# Autodesk Inventor assembly: Tête
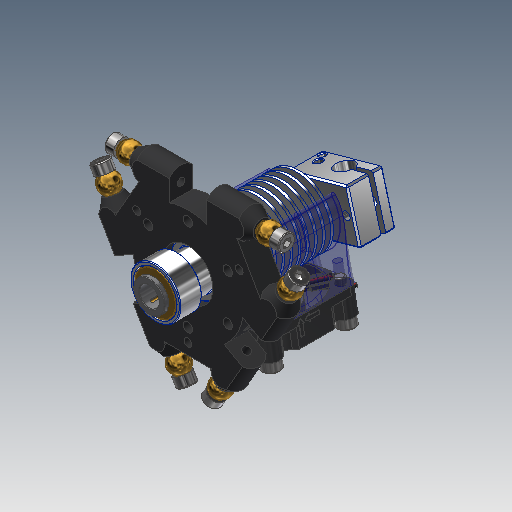
[picture p0: Inventor's stored thumbnail of the model, 512x512]
Saved by Autodesk Inventor 2017 (Build 210142000, 142)
## iProperties
Company: FABLAB Frenchmakers
Part Number: Tête
Material: Générique
Document SubType Name: Assembly
Designer: FABLAB Frenchmakers
Mass: 87.2442 g
Surface Area: 323.979 cm^2
Volume: 30.3794 cm^3
Density: 2.87182 g/cm^3
Project: 1420 Vauban 3D XL
Catalog Web Link: http://frenchmakers.com/
Stock Number: 1420-02-00
## Documents named in this file (8)
- W:\Professionnel\Conception FABLAB\1420-Vauban 3D XL\1420-02 Tete\1420-02-00 Tete.iam
- W:\Professionnel\Conception FABLAB\1420-Vauban 3D XL\1420-02 Tete\1420-02-01 Efflector.ipt
- Support_buse.ipt
- W:\Professionnel\Conception FABLAB\1420-Vauban 3D XL\1420-02 Tete\1420-02-04 Rotule.ipt
- W:\Professionnel\Conception FABLAB\1420-Vauban 3D XL\1420-90 Centre de contenu\fr-FR\ANSI B18.3.1M(1)\ANSI B18.3.1M - M3x0,5 x 10(2).ipt
- W:\Professionnel\Conception FABLAB\1420-Vauban 3D XL\1420-02 Tete\Buse_E3D_V6\1420-02-20 Buse E3d V6.iam
- W:\Professionnel\Conception FABLAB\1420-Vauban 3D XL\1420-02 Tete\1420-02-02 Support ventillateur E3D.ipt
- W:\Professionnel\Conception FABLAB\1420-Vauban 3D XL\1420-02 Tete\1420-02-03 Ventilateur 30x30.ipt
## Components (20 placed, 6 different names)
1. 1420-02-20 Buse E3d V6:1 [sub-assembly] — Placage:25, Affleurement:1, Placage:26
2. Support_buse:1 — Placage:1, Placage:2, Placage:3, Placage:4, Placage:5, Placage:6, Placage:7, Placage:8, Placage:9, Placage:10, Placage:11, Placage:12, Placage:25, Affleurement:1, Placage:27
3. Vis à tête percée - Métrique M3x0,5 x 10:1 — Placage:13, Placage:23
4. Vis à tête percée - Métrique M3x0,5 x 10:2 — Placage:14, Placage:24
5. Vis à tête percée - Métrique M3x0,5 x 10:3 — Placage:15, Placage:22
6. Vis à tête percée - Métrique M3x0,5 x 10:4 — Placage:16, Placage:21
7. Vis à tête percée - Métrique M3x0,5 x 10:5 — Placage:17, Placage:19
8. Vis à tête percée - Métrique M3x0,5 x 10:6 — Placage:18, Placage:20
9. 1420-02-04 Rotule:1 — Placage:3, Placage:8, Placage:16, Placage:21
10. 1420-02-04 Rotule:2 — Placage:4, Placage:7, Placage:15, Placage:22
11. 1420-02-04 Rotule:3 — Placage:5, Placage:12, Placage:13, Placage:23
12. 1420-02-04 Rotule:4 — Placage:6, Placage:11, Placage:14, Placage:24
13. 1420-02-04 Rotule:5 — Placage:1, Placage:10, Placage:17, Placage:19
14. 1420-02-04 Rotule:6 — Placage:2, Placage:9, Placage:18, Placage:20
15. 1420-02-02 Support ventillateur E3D:1 — Placage:26, Placage:27, Placage:28, Placage:29, Placage:30
16. 1420-02-03 Ventilateur 30x30:1 — Placage:28, Placage:29, Placage:30, Placage:31, Placage:32, Placage:33, Placage:34, Placage:35
17. Vis à tête percée - Métrique M3x0,5 x 10:7 — Affleurement:2, Placage:31
18. Vis à tête percée - Métrique M3x0,5 x 10:8 — Affleurement:2, Affleurement:3, Placage:32
19. Vis à tête percée - Métrique M3x0,5 x 10:9 — Affleurement:3, Affleurement:4, Placage:34, Placage:35
20. Vis à tête percée - Métrique M3x0,5 x 10:10 — Affleurement:4, Placage:33
## Relationships (39: Mate 35, Flush 4)
- Placage:1 [Mate]: Support_buse:1 ↔ 1420-02-04 Rotule:5
- Placage:2 [Mate]: Support_buse:1 ↔ 1420-02-04 Rotule:6
- Placage:3 [Mate]: Support_buse:1 ↔ 1420-02-04 Rotule:1
- Placage:4 [Mate]: Support_buse:1 ↔ 1420-02-04 Rotule:2
- Placage:5 [Mate]: Support_buse:1 ↔ 1420-02-04 Rotule:3
- Placage:6 [Mate]: Support_buse:1 ↔ 1420-02-04 Rotule:4
- Placage:7 [Mate]: Support_buse:1 ↔ 1420-02-04 Rotule:2
- Placage:8 [Mate]: Support_buse:1 ↔ 1420-02-04 Rotule:1
- Placage:9 [Mate]: Support_buse:1 ↔ 1420-02-04 Rotule:6
- Placage:10 [Mate]: Support_buse:1 ↔ 1420-02-04 Rotule:5
- Placage:11 [Mate]: Support_buse:1 ↔ 1420-02-04 Rotule:4
- Placage:12 [Mate]: Support_buse:1 ↔ 1420-02-04 Rotule:3
- Placage:13 [Mate]: Vis à tête percée - Métrique M3x0,5 x 10:1 ↔ 1420-02-04 Rotule:3
- Placage:14 [Mate]: Vis à tête percée - Métrique M3x0,5 x 10:2 ↔ 1420-02-04 Rotule:4
- Placage:15 [Mate]: Vis à tête percée - Métrique M3x0,5 x 10:3 ↔ 1420-02-04 Rotule:2
- Placage:16 [Mate]: Vis à tête percée - Métrique M3x0,5 x 10:4 ↔ 1420-02-04 Rotule:1
- Placage:17 [Mate]: Vis à tête percée - Métrique M3x0,5 x 10:5 ↔ 1420-02-04 Rotule:5
- Placage:18 [Mate]: Vis à tête percée - Métrique M3x0,5 x 10:6 ↔ 1420-02-04 Rotule:6
- Placage:19 [Mate]: Vis à tête percée - Métrique M3x0,5 x 10:5 ↔ 1420-02-04 Rotule:5
- Placage:20 [Mate]: Vis à tête percée - Métrique M3x0,5 x 10:6 ↔ 1420-02-04 Rotule:6
- Placage:21 [Mate]: Vis à tête percée - Métrique M3x0,5 x 10:4 ↔ 1420-02-04 Rotule:1
- Placage:22 [Mate]: Vis à tête percée - Métrique M3x0,5 x 10:3 ↔ 1420-02-04 Rotule:2
- Placage:23 [Mate]: Vis à tête percée - Métrique M3x0,5 x 10:1 ↔ 1420-02-04 Rotule:3
- Placage:24 [Mate]: Vis à tête percée - Métrique M3x0,5 x 10:2 ↔ 1420-02-04 Rotule:4
- Placage:25 [Mate]: 1420-02-20 Buse E3d V6:1 ↔ Support_buse:1
- Affleurement:1 [Flush] (10.5 mm): 1420-02-20 Buse E3d V6:1 ↔ Support_buse:1
- Placage:26 [Mate]: 1420-02-20 Buse E3d V6:1 ↔ 1420-02-02 Support ventillateur E3D:1
- Placage:27 [Mate]: Support_buse:1 ↔ 1420-02-02 Support ventillateur E3D:1
- Placage:28 [Mate]: 1420-02-02 Support ventillateur E3D:1 ↔ 1420-02-03 Ventilateur 30x30:1
- Placage:29 [Mate]: 1420-02-02 Support ventillateur E3D:1 ↔ 1420-02-03 Ventilateur 30x30:1
- Placage:30 [Mate]: 1420-02-02 Support ventillateur E3D:1 ↔ 1420-02-03 Ventilateur 30x30:1
- Affleurement:2 [Flush]: Vis à tête percée - Métrique M3x0,5 x 10:7 ↔ Vis à tête percée - Métrique M3x0,5 x 10:8
- Affleurement:3 [Flush]: Vis à tête percée - Métrique M3x0,5 x 10:8 ↔ Vis à tête percée - Métrique M3x0,5 x 10:9
- Affleurement:4 [Flush]: Vis à tête percée - Métrique M3x0,5 x 10:9 ↔ Vis à tête percée - Métrique M3x0,5 x 10:10
- Placage:31 [Mate]: 1420-02-03 Ventilateur 30x30:1 ↔ Vis à tête percée - Métrique M3x0,5 x 10:7
- Placage:32 [Mate]: 1420-02-03 Ventilateur 30x30:1 ↔ Vis à tête percée - Métrique M3x0,5 x 10:8
- Placage:33 [Mate]: 1420-02-03 Ventilateur 30x30:1 ↔ Vis à tête percée - Métrique M3x0,5 x 10:10
- Placage:34 [Mate]: 1420-02-03 Ventilateur 30x30:1 ↔ Vis à tête percée - Métrique M3x0,5 x 10:9
- Placage:35 [Mate]: 1420-02-03 Ventilateur 30x30:1 ↔ Vis à tête percée - Métrique M3x0,5 x 10:9
